# Autodesk Inventor assembly: ensamble_general
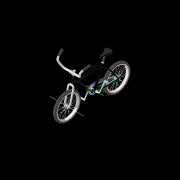
[picture p0: Inventor's stored thumbnail of the model, 180x180]
Saved by Autodesk Inventor 2021 (Build 250183000, 183)
## iProperties
Created: 2021-04-10
Part Number: ensamble_general
Document SubType Name: Assembly
Designer: j2seb
Author: j2seb
## Documents named in this file (9)
- C:\Users\maaro\Documents\UNAL\Automatización de Procesos de Manufactura\Github\Proyecto_APM\02 Inventor\ensamble_general.iam
- G:\Unidades compartidas\APM\02 Inventor-Drive\Marco_Bicicleta.iam
- G:\Unidades compartidas\APM\02 Inventor-Drive\Manubrio\Manubrio.ipt
- G:\Unidades compartidas\APM\02 Inventor-Drive\sillin.iam
- G:\Unidades compartidas\APM\02 Inventor-Drive\caja_pedalera.iam
- G:\Unidades compartidas\APM\02 Inventor-Drive\Transmision\Cadena.iam
- G:\Unidades compartidas\APM\02 Inventor-Drive\cubrecadena.ipt
- G:\Unidades compartidas\APM\02 Inventor-Drive\llanta trasera.iam
- C:\Users\maaro\Documents\UNAL\Automatización de Procesos de Manufactura\Github\Proyecto_APM\02 Inventor\llanta delantera.iam
## Components (8 placed, 8 different names)
1. Marco_Bicicleta:1 [sub-assembly] — Flush:1, Cylindrical:2, Mate:5, Coincidencia:6, Coincidencia:7, Mate:8, Mate:9, Coincidencia:16, Coincidencia:19, Mate:20
2. Manubrio:1 — Flush:1, Coincidencia:19, Mate:21
3. sillin:1 [sub-assembly] — Cylindrical:2, Mate:5
4. caja_pedalera:1 [sub-assembly] — Coincidencia:6, Coincidencia:7
5. Cadena:1 [sub-assembly] — Mate:12
6. cubrecadena:1 — Mate:15
7. llanta trasera:1 [sub-assembly] — Coincidencia:16
8. llanta delantera:1 [sub-assembly] — Mate:20, Mate:22
## Relationships (15: Mate 13, Flush 1, CylindricalJoint 1)
- [Mate]: Marco_Bicicleta:1 ↔ llanta trasera:1
- Flush:1 (-55.052 mm): Marco_Bicicleta:1 ↔ Manubrio:1
- Cylindrical:2: Marco_Bicicleta:1 ↔ sillin:1
- Mate:5 (-50 mm): Marco_Bicicleta:1 ↔ sillin:1
- Coincidencia:6 [Mate]: Marco_Bicicleta:1 ↔ caja_pedalera:1
- Coincidencia:7 [Mate]: Marco_Bicicleta:1 ↔ caja_pedalera:1
- Mate:8: Marco_Bicicleta:1
- Mate:9: Marco_Bicicleta:1
- Mate:12: Cadena:1
- Mate:15: cubrecadena:1
- Coincidencia:16 [Mate]: Marco_Bicicleta:1 ↔ llanta trasera:1
- Coincidencia:19 [Mate]: Marco_Bicicleta:1 ↔ Manubrio:1
- Mate:20: Marco_Bicicleta:1 ↔ llanta delantera:1
- Mate:21: Manubrio:1
- Mate:22: llanta delantera:1
## Named parameters: DExtTub = 42.164 mm, DintTub = 35.052 mm, DIntTubTen = 28 mm, DAguUniMarcoLlanta = 5 mm
